# Autodesk Inventor assembly: CRA-ASM-1003
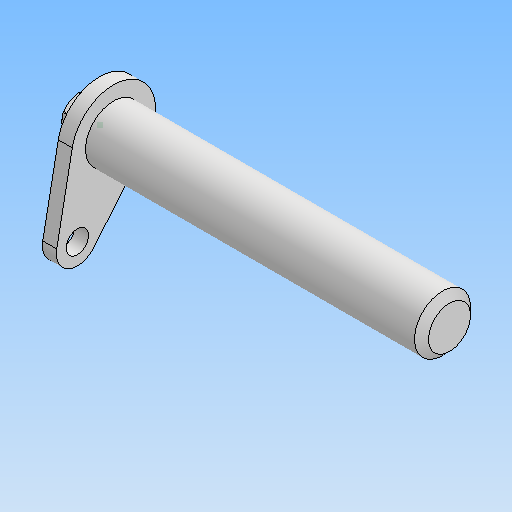
[picture p0: Inventor's stored thumbnail of the model, 512x512]
Saved by Autodesk Inventor 2025.4 (Build 294407000, 407)
## iProperties
Created: 2025-12-20
Part Number: CRA-ASM-1003
Description: CLEANING ARM CAGE PIVOT PIN ASSEMBLY
Document SubType Name: Assembly
Designer: josh
Mass: 182.574 g
Surface Area: 204.509 cm^2
Volume: 89.1634 cm^3
Density: 2.04763 g/cm^3
Author: josh
## iProperties of the stored document MemberDocs/xT1i43wx1Cs5yguycZihf1q2p2a
Created: 2025-12-20
Part Number: CRA-ASM-1003
Description: CLEANING ARM CAGE PIVOT PIN ASSEMBLY
Document SubType Name: Assembly
Designer: josh
Mass: 182.574 g
Surface Area: 204.509 cm^2
Volume: 89.1634 cm^3
Density: 2.04763 g/cm^3
Author: josh
## Documents named in this file (4)
- R:\A1- Neuweg Design Data\OM Robotics\CLEANING ROBOT TOWER PROJECT\CRA-ASM-1003.iam
- R:\A1- Neuweg Design Data\OM Robotics\CLEANING ROBOT TOWER PROJECT\CRA-1025.ipt
- R:\A1- Neuweg Design Data\OM Robotics\CLEANING ROBOT TOWER PROJECT\CRA-1026.ipt
- R:\A1- Neuweg Design Data\OM Robotics\CLEANING ROBOT TOWER PROJECT\92979A340.ipt
## Components (3 placed, 3 different names)
1. CRA-1026:1
2. CRA-1025:1 — Insert:1
3. 92979A340:1 — Insert:1
## Relationships (1: Insert 1)
- Insert:1: CRA-1025:1 ↔ 92979A340:1
